# Autodesk Inventor assembly: 2.75 Omni AS, No Insert-back-left-back-right
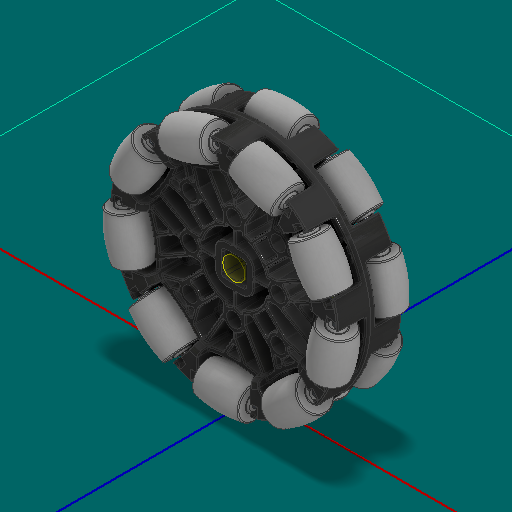
[picture p0: Inventor's stored thumbnail of the model, 512x512]
Saved by Autodesk Inventor 2025 (Build 290162000, 162)
## iProperties
Created: 2022-08-02
Part Number: 2.75 Omni AS, No Insert-back-left-back-right
Document SubType Name: Assembly
Designer: averey
Author: ylu12
## Documents named in this file (2)
- C:\Users\avere\rbp_cad\atlas\chassis\drive-pod-back-right\2.75 Omni AS, No Insert-back-left-back-right.iam
- C:\Users\avere\rbp_cad\atlas\chassis\drive-pod-back-right\2.75 Omni Antistatic-back-left-back-right.ipt
## Components (1 placed, 1 different names)
1. 2.75 Omni Antistatic-back-left-back-right:1 — Flush:4, Mate:7, Mate:8
## Relationships (3: Mate 2, Flush 1)
- Flush:4: 2.75 Omni Antistatic-back-left-back-right:1
- Mate:7: 2.75 Omni Antistatic-back-left-back-right:1
- Mate:8: 2.75 Omni Antistatic-back-left-back-right:1
